# Autodesk Inventor assembly: ASM Frame
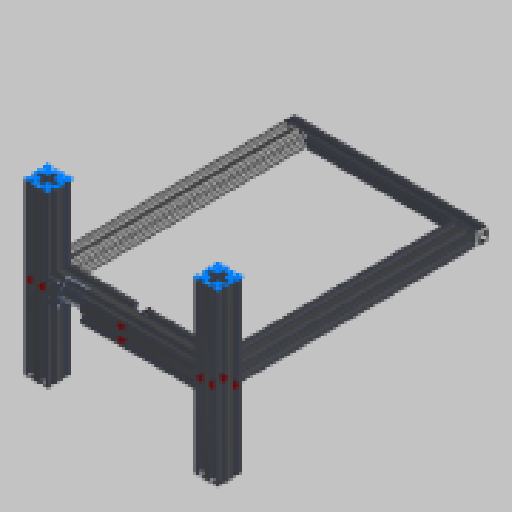
[picture p0: Inventor's stored thumbnail of the model, 512x512]
Saved by Autodesk Inventor 2025.4 (Build 294407000, 407)
## iProperties
Created: 2022-04-13
Part Number: ASM Frame
Document SubType Name: Assembly
Designer: javie
Author: javie
Revision Number: ANY
## Documents named in this file (8)
- C:\Users\Inema\OneDrive - INEMA S.A\Escritorio\Modelo Ender 3\ASM Frame.iam
- C:\Users\Inema\OneDrive - INEMA S.A\Escritorio\Modelo Ender 3\4040 profile.ipt
- C:\Users\Inema\OneDrive - INEMA S.A\Escritorio\Modelo Ender 3\4040-3 profile.ipt
- C:\Users\Inema\OneDrive - INEMA S.A\Escritorio\Modelo Ender 3\2020-2 profile.ipt
- C:\Users\Inema\OneDrive - INEMA S.A\Escritorio\Modelo Ender 3\2040-3R profile.ipt
- C:\Users\Inema\OneDrive - INEMA S.A\Escritorio\Modelo Ender 3\2040-3L profile.ipt
- C:\Users\Inema\OneDrive - INEMA S.A\Escritorio\Modelo Ender 3\2020 Endcap.ipt
- C:\Users\Inema\OneDrive - INEMA S.A\Escritorio\Modelo Ender 3\M5X45 Socket Head Screw.ipt
## Components (30 placed, 30 different names)
1. 4040 profile_265
2. 4040 profile_266
3. 4040-3 profile_267
4. 2020-2 profile_268 — Coincidencia:1, Nivelación:1, Nivelación:2
5. 2040-3R profile_269
6. 2040-3L profile_270
7. 2020 Endcap_272
8. 2020 Endcap_273
9. 2020 Endcap_274
10. M5X45 Socket Head Screw_275
11. M5X45 Socket Head Screw_276
12. M5X45 Socket Head Screw_277
13. M5X45 Socket Head Screw_278
14. M5X45 Socket Head Screw_279
15. M5X45 Socket Head Screw_280
16. M5X45 Socket Head Screw_281
17. M5X45 Socket Head Screw_282
18. M5X45 Socket Head Screw_283
19. M5X45 Socket Head Screw_284
20. M5X45 Socket Head Screw_285
21. M5X45 Socket Head Screw_286
22. M5X45 Socket Head Screw_287
23. M5X45 Socket Head Screw_288
24. 2020 Endcap_289
25. 2020 Endcap_290
26. 2020 Endcap_291
27. 2020 Endcap_292
28. 2020 Endcap_293
29. 2020 Endcap_294
30. 2020 Endcap:11 — Coincidencia:1, Nivelación:1, Nivelación:2
## Relationships (3: Flush 2, Mate 1)
- Coincidencia:1 [Mate]: 2020-2 profile_268 ↔ 2020 Endcap:11
- Nivelación:1 [Flush]: 2020-2 profile_268 ↔ 2020 Endcap:11
- Nivelación:2 [Flush]: 2020-2 profile_268 ↔ 2020 Endcap:11
